# Autodesk Inventor assembly: secondVersion
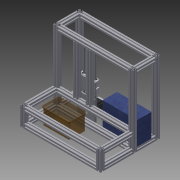
[picture p0: Inventor's stored thumbnail of the model, 180x180]
Saved by Autodesk Inventor 2015 SP1 (Build 190203100, 203)
## iProperties
Created: 2015-07-17
Part Number: secondVersion
Document SubType Name: Assembly
Designer: ubik
Author: ubik
## Documents named in this file (17)
- C:\Users\ubik\Dropbox\DueTech\cable test\secondVersion.iam
- C:\Users\ubik\Dropbox\DueTech\cable test\cuva.ipt
- C:\Users\ubik\Dropbox\DueTech\cable test\20.1068-30X30-3.ipt
- C:\Users\ubik\Dropbox\DueTech\cable test\20.1068-30X30-3\20.1068-30X30-200.ipt
- C:\Users\ubik\Dropbox\DueTech\cable test\20.1068-30X30-3\20.1068-30X30-130.ipt
- C:\Users\ubik\Dropbox\DueTech\cable test\alu top plate.ipt
- C:\Users\ubik\Dropbox\proiecte\inventor\inventor library\sk12.ipt
- C:\Users\ubik\Dropbox\DueTech\cable test\linear shaft.ipt
- C:\Users\ubik\Dropbox\DueTech\cable test\linear shaft\Shaft 12 450.ipt
- C:\Users\ubik\Dropbox\proiecte\inventor\inventor library\sc12uu\SCS12UU.iam
- C:\Users\ubik\Dropbox\DueTech\cable test\mobile plate.ipt
- C:\Users\ubik\Dropbox\proiecte\inventor\inventor library\57BYGH311D-12\57BYGH311D-12.iam
- C:\Users\ubik\Dropbox\DueTech\cable test\motor plate support.ipt
- C:\Users\ubik\Dropbox\DueTech\cable test\20.1068-30X30-3\20.1068-30X30-340.ipt
- C:\Users\ubik\Dropbox\DueTech\cable test\20.1068-30X30-3\20.1068-30X30-500.ipt
- C:\Users\ubik\Dropbox\DueTech\cable test\pompa.ipt
- C:\Users\ubik\Dropbox\DueTech\cable test\clema cablu profil.ipt
## Components (40 placed, 14 different names)
1. cuva:1 — Flush:73
2. 20.1068-30X30-500:2 — Mate:11, Flush:18, Flush:19, Flush:23, Mate:12, Flush:63, Mate:47
3. 20.1068-30X30-500:3 — Flush:6, Flush:7, Mate:2, Flush:12, Mate:8, Flush:13, Flush:17, Flush:73
4. 20.1068-30X30-500:4 — Mate:13, Flush:25, Flush:26, Flush:67
5. 20.1068-30X30-200:5 — Flush:20, Flush:21, Flush:24
6. 20.1068-30X30-200:6 — Mate:10, Flush:16, Flush:17, Flush:85
7. 20.1068-30X30-200:7 — Flush:4, Mate:1, Flush:5, Flush:9, Mate:3
8. 20.1068-30X30-200:8 — Flush:20, Flush:21, Flush:22, Flush:23, Mate:12, Flush:25, Flush:54
9. 20.1068-30X30-130:9 — Flush:4, Mate:1, Flush:5, Flush:6, Flush:7, Mate:2, Mate:13
10. 20.1068-30X30-500:10 — Flush:9, Mate:3, Flush:22, Flush:66, Mate:44, Flush:69, Flush:70, Mate:52, Flush:79, Flush:80, Mate:55, Flush:87
11. 20.1068-30X30-500:11 — Mate:11, Flush:18, Flush:19, Flush:24, Flush:74, Mate:49, Flush:77, Mate:51, Flush:78, Flush:86
12. 20.1068-30X30-130:12 — Flush:12, Mate:8, Flush:13, Mate:10, Flush:16, Flush:26, Flush:67
13. 20.1068-30X30-340:13 — Flush:27, Flush:28, Mate:15, Mate:16, Flush:30, Flush:31
14. 20.1068-30X30-340:14 — Flush:27, Flush:28, Mate:15
15. alu top plate:1 — Mate:16, Flush:30, Flush:31, Mate:17, Mate:18, Mate:19, Mate:20
16. sk12:1 — Flush:32, Flush:33, Flush:36, Flush:38, Mate:17, Mate:18, Mate:20, Mate:22, Flush:40
17. sk12:2 — Flush:32, Flush:33, Flush:37, Mate:19, Mate:21
18. sk12:3 — Flush:34, Flush:35, Flush:36, Flush:37, Mate:42
19. sk12:4 — Flush:34, Flush:35, Flush:38, Mate:30, Mate:40, Mate:41
20. Shaft 12 450:1 — Flush:39, Mate:22, Flush:40, Mate:23, Mate:25
21. Shaft 12 450:2 — Flush:39, Mate:21, Mate:24
22. SCS12UU:1 [sub-assembly] — Flush:41, Flush:43, Flush:44, Mate:23, Mate:26
23. SCS12UU:2 [sub-assembly] — Flush:42, Flush:43, Flush:44, Mate:24
24. SCS12UU:3 [sub-assembly] — Flush:42, Flush:45, Flush:46, Mate:28, Mate:29
25. SCS12UU:4 [sub-assembly] — Flush:41, Flush:45, Flush:46, Mate:25, Mate:27
26. mobile plate:1 — Mate:26, Mate:27, Mate:28, Mate:29
27. 57BYGH311D-12:1 [sub-assembly] — Mate:32, Mate:33
28. motor plate support:1 — Mate:30, Mate:32, Mate:33, Mate:40, Mate:41, Mate:42, Flush:63
29. 20.1068-30X30-130:16 — Flush:54, Mate:37, Flush:64, Mate:43, Flush:65, Flush:66, Mate:47
30. 20.1068-30X30-500:20 — Mate:37, Flush:68, Mate:48, Flush:75, Mate:50, Flush:76, Flush:84
31. 20.1068-30X30-500:22 — Flush:64, Mate:43, Flush:65, Flush:68, Flush:81, Mate:53
32. 20.1068-30X30-130:23 — Mate:44, Flush:69, Flush:70
33. pompa:1 — Flush:74, Mate:48, Mate:49
34. 20.1068-30X30-130:27 — Flush:77, Mate:51, Flush:78
35. 20.1068-30X30-500:29 — Flush:75, Mate:50, Flush:76, Flush:82, Mate:54, Flush:83
36. 20.1068-30X30-500:30 — Flush:81, Mate:53, Flush:82
37. 20.1068-30X30-500:31 — Mate:52, Flush:79, Flush:80
38. 20.1068-30X30-130:32 — Mate:54, Flush:83, Flush:84
39. 20.1068-30X30-500:33 — Mate:55, Flush:85, Flush:86
40. clema cablu profil:1 — Flush:87
## Relationships (102: Flush 61, Mate 41)
- Flush:4: 20.1068-30X30-200:7 ↔ 20.1068-30X30-130:9
- Mate:1: 20.1068-30X30-200:7 ↔ 20.1068-30X30-130:9
- Flush:5: 20.1068-30X30-200:7 ↔ 20.1068-30X30-130:9
- Flush:6: 20.1068-30X30-500:3 ↔ 20.1068-30X30-130:9
- Flush:7: 20.1068-30X30-500:3 ↔ 20.1068-30X30-130:9
- Mate:2: 20.1068-30X30-500:3 ↔ 20.1068-30X30-130:9
- Flush:9: 20.1068-30X30-200:7 ↔ 20.1068-30X30-500:10
- Mate:3: 20.1068-30X30-200:7 ↔ 20.1068-30X30-500:10
- Flush:12: 20.1068-30X30-500:3 ↔ 20.1068-30X30-130:12
- Mate:8: 20.1068-30X30-500:3 ↔ 20.1068-30X30-130:12
- Flush:13: 20.1068-30X30-500:3 ↔ 20.1068-30X30-130:12
- Mate:10: 20.1068-30X30-200:6 ↔ 20.1068-30X30-130:12
- Flush:16: 20.1068-30X30-200:6 ↔ 20.1068-30X30-130:12
- Flush:17: 20.1068-30X30-500:3 ↔ 20.1068-30X30-200:6
- Mate:11: 20.1068-30X30-500:2 ↔ 20.1068-30X30-500:11
- Flush:18: 20.1068-30X30-500:2 ↔ 20.1068-30X30-500:11
- Flush:19: 20.1068-30X30-500:2 ↔ 20.1068-30X30-500:11
- Flush:20: 20.1068-30X30-200:5 ↔ 20.1068-30X30-200:8
- Flush:21: 20.1068-30X30-200:5 ↔ 20.1068-30X30-200:8
- Flush:22: 20.1068-30X30-200:8 ↔ 20.1068-30X30-500:10
- Flush:23: 20.1068-30X30-500:2 ↔ 20.1068-30X30-200:8
- Mate:12: 20.1068-30X30-500:2 ↔ 20.1068-30X30-200:8
- Flush:24: 20.1068-30X30-200:5 ↔ 20.1068-30X30-500:11
- Mate:13: 20.1068-30X30-500:4 ↔ 20.1068-30X30-130:9
- Flush:25: 20.1068-30X30-500:4 ↔ 20.1068-30X30-200:8
- Flush:26: 20.1068-30X30-500:4 ↔ 20.1068-30X30-130:12
- Flush:27: 20.1068-30X30-340:13 ↔ 20.1068-30X30-340:14
- Flush:28: 20.1068-30X30-340:13 ↔ 20.1068-30X30-340:14
- Mate:15 (60 mm): 20.1068-30X30-340:13 ↔ 20.1068-30X30-340:14
- Mate:16: 20.1068-30X30-340:13 ↔ alu top plate:1
- Flush:30: 20.1068-30X30-340:13 ↔ alu top plate:1
- Flush:31: 20.1068-30X30-340:13 ↔ alu top plate:1
- Flush:32: sk12:1 ↔ sk12:2
- Flush:33: sk12:1 ↔ sk12:2
- Flush:34: sk12:3 ↔ sk12:4
- Flush:35: sk12:3 ↔ sk12:4
- Flush:36: sk12:1 ↔ sk12:3
- Flush:37: sk12:2 ↔ sk12:3
- Flush:38: sk12:1 ↔ sk12:4
- Mate:17: alu top plate:1 ↔ sk12:1
- Mate:18: alu top plate:1 ↔ sk12:1
- Mate:19: alu top plate:1 ↔ sk12:2
- Mate:20: alu top plate:1 ↔ sk12:1
- Flush:39: Shaft 12 450:1 ↔ Shaft 12 450:2
- Mate:21: sk12:2 ↔ Shaft 12 450:2
- Mate:22: sk12:1 ↔ Shaft 12 450:1
- Flush:40: sk12:1 ↔ Shaft 12 450:1
- Flush:41: SCS12UU:1 ↔ SCS12UU:4
- Flush:42: SCS12UU:2 ↔ SCS12UU:3
- Flush:43: SCS12UU:1 ↔ SCS12UU:2
- Flush:44: SCS12UU:1 ↔ SCS12UU:2
- Flush:45: SCS12UU:3 ↔ SCS12UU:4
- Flush:46: SCS12UU:3 ↔ SCS12UU:4
- Mate:23: Shaft 12 450:1 ↔ SCS12UU:1
- Mate:24: Shaft 12 450:2 ↔ SCS12UU:2
- Mate:25: Shaft 12 450:1 ↔ SCS12UU:4
- Mate:26: SCS12UU:1 ↔ mobile plate:1
- Mate:27: SCS12UU:4 ↔ mobile plate:1
- Mate:28: SCS12UU:3 ↔ mobile plate:1
- Mate:29: SCS12UU:3 ↔ mobile plate:1
- Mate:30: sk12:4 ↔ motor plate support:1
- Mate:32: 57BYGH311D-12:1 ↔ motor plate support:1
- Mate:33 (25 mm): 57BYGH311D-12:1 ↔ motor plate support:1
- Flush:54: 20.1068-30X30-200:8 ↔ 20.1068-30X30-130:16
- Mate:37: 20.1068-30X30-130:16 ↔ 20.1068-30X30-500:20
- Mate:40: sk12:4 ↔ motor plate support:1
- Mate:41: sk12:4 ↔ motor plate support:1
- Mate:42: sk12:3 ↔ motor plate support:1
- Flush:63: 20.1068-30X30-500:2 ↔ motor plate support:1
- Flush:64: 20.1068-30X30-130:16 ↔ 20.1068-30X30-500:22
- Mate:43: 20.1068-30X30-130:16 ↔ 20.1068-30X30-500:22
- Flush:65: 20.1068-30X30-130:16 ↔ 20.1068-30X30-500:22
- Flush:66: 20.1068-30X30-500:10 ↔ 20.1068-30X30-130:16
- Flush:67: 20.1068-30X30-500:4 ↔ 20.1068-30X30-130:12
- Flush:68: 20.1068-30X30-500:20 ↔ 20.1068-30X30-500:22
- Mate:44: 20.1068-30X30-500:10 ↔ 20.1068-30X30-130:23
- Flush:69: 20.1068-30X30-500:10 ↔ 20.1068-30X30-130:23
- Flush:70: 20.1068-30X30-500:10 ↔ 20.1068-30X30-130:23
- Mate:47: 20.1068-30X30-500:2 ↔ 20.1068-30X30-130:16
- Flush:73: cuva:1 ↔ 20.1068-30X30-500:3
- Flush:74: 20.1068-30X30-500:11 ↔ pompa:1
- Mate:48: 20.1068-30X30-500:20 ↔ pompa:1
- Mate:49: 20.1068-30X30-500:11 ↔ pompa:1
- Flush:75: 20.1068-30X30-500:20 ↔ 20.1068-30X30-500:29
- Mate:50: 20.1068-30X30-500:20 ↔ 20.1068-30X30-500:29
- Flush:76: 20.1068-30X30-500:20 ↔ 20.1068-30X30-500:29
- Flush:77: 20.1068-30X30-500:11 ↔ 20.1068-30X30-130:27
- Mate:51: 20.1068-30X30-500:11 ↔ 20.1068-30X30-130:27
- Flush:78: 20.1068-30X30-500:11 ↔ 20.1068-30X30-130:27
- Mate:52: 20.1068-30X30-500:10 ↔ 20.1068-30X30-500:31
- Flush:79: 20.1068-30X30-500:10 ↔ 20.1068-30X30-500:31
- Flush:80: 20.1068-30X30-500:10 ↔ 20.1068-30X30-500:31
- Flush:81: 20.1068-30X30-500:22 ↔ 20.1068-30X30-500:30
- Mate:53: 20.1068-30X30-500:22 ↔ 20.1068-30X30-500:30
- Flush:82: 20.1068-30X30-500:29 ↔ 20.1068-30X30-500:30
- Mate:54: 20.1068-30X30-500:29 ↔ 20.1068-30X30-130:32
- Flush:83: 20.1068-30X30-500:29 ↔ 20.1068-30X30-130:32
- Flush:84: 20.1068-30X30-500:20 ↔ 20.1068-30X30-130:32
- Mate:55: 20.1068-30X30-500:10 ↔ 20.1068-30X30-500:33
- Flush:85: 20.1068-30X30-200:6 ↔ 20.1068-30X30-500:33
- Flush:86: 20.1068-30X30-500:11 ↔ 20.1068-30X30-500:33
- Flush:87: 20.1068-30X30-500:10 ↔ clema cablu profil:1
